# Autodesk Inventor assembly: sholder
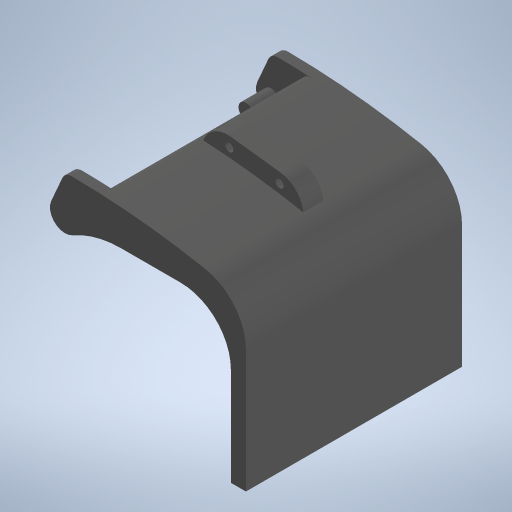
[picture p0: Inventor's stored thumbnail of the model, 512x512]
Saved by Autodesk Inventor 2024.1 (Build 281209000, 209)
## iProperties
Created: 2024-10-17
Part Number: sholder
Document SubType Name: Assembly
Designer: hibik
Author: hibik
## Documents named in this file (3)
- C:\Users\hibik\Documents\Robomech\HR\Eglantyne\hard\arm\sholder.iam
- C:\Users\hibik\Documents\Robomech\HR\Eglantyne\hard\arm\sholder.ipt
- C:\Users\hibik\Documents\Robomech\HR\Eglantyne\hard\arm\sholder_2.ipt
## Components (2 placed, 2 different names)
1. sholder:1 — 挿入:1, 挿入:2
2. sholder_2:1 — 挿入:1, 挿入:2
## Relationships (2: Insert 2)
- 挿入:1 [Insert]: sholder:1 ↔ sholder_2:1
- 挿入:2 [Insert]: sholder:1 ↔ sholder_2:1
